# Autodesk Inventor assembly: one_wheel
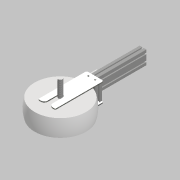
[picture p0: Inventor's stored thumbnail of the model, 180x180]
Saved by Autodesk Inventor 2021.2 (Build 252289000, 289)
## iProperties
Created: 2021-05-27
Part Number: one_wheel
Document SubType Name: Assembly
Designer: gisen
Author: gisen
## Documents named in this file (4)
- C:\Users\gisen\workspace\beetle_inventor_model\suspension\rocker.iam
- C:\Users\gisen\workspace\beetle_inventor_model\suspension\wheel_with_mounts.iam
- C:\Users\gisen\workspace\beetle_inventor_model\suspension\wheel_frame_mount.ipt
- C:\Users\gisen\workspace\beetle_inventor_model\suspension\AFS-2040-4-150.ipt
## Components (3 placed, 3 different names)
1. wheel_with_mounts:1 [sub-assembly] — フラッシュ:1, メイト:1, メイト:2, メイト:5
2. AFS-2040-4-150:1 — フラッシュ:1, メイト:1, メイト:2, メイト:3, メイト:4, メイト:6
3. wheel_frame_mount:1 — メイト:3, メイト:4, メイト:5, メイト:6
## Relationships (7: Mate 6, Flush 1)
- フラッシュ:1 [Flush]: wheel_with_mounts:1 ↔ AFS-2040-4-150:1
- メイト:1 [Mate]: wheel_with_mounts:1 ↔ AFS-2040-4-150:1
- メイト:2 [Mate]: wheel_with_mounts:1 ↔ AFS-2040-4-150:1
- メイト:3 [Mate]: AFS-2040-4-150:1 ↔ wheel_frame_mount:1
- メイト:4 [Mate] (-10 mm): AFS-2040-4-150:1 ↔ wheel_frame_mount:1
- メイト:5 [Mate] (-10 mm): wheel_with_mounts:1 ↔ wheel_frame_mount:1
- メイト:6 [Mate] (-10 mm): AFS-2040-4-150:1 ↔ wheel_frame_mount:1
